# Autodesk Inventor assembly: Thrust_Duct
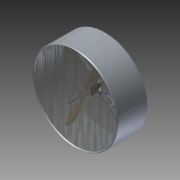
[picture p0: Inventor's stored thumbnail of the model, 180x180]
Saved by Autodesk Inventor 2011 SP1 (Build 150282100, 282)
## iProperties
Created: 2011-06-11
Part Number: Thrust_Duct
Document SubType Name: Assembly
Designer: Andrew G. Meyer
Mass: 210.395 g
Surface Area: 2926.53 cm^2
Volume: 210.395 cm^3
Density: 1 g/cm^3
Author: Andrew G. Meyer
## Documents named in this file (9)
- C:\Users\Andrew G. Meyer\Documents\Inventor\Hovercraft\Thrust_Duct.iam
- C:\Users\Andrew G. Meyer\Documents\Inventor\Hovercraft\Duct_Inner.ipt
- C:\Users\Andrew G. Meyer\Documents\Inventor\Hovercraft\Duct_Outer.ipt
- C:\Users\Andrew G. Meyer\Documents\Inventor\Hovercraft\Thrust_Support.ipt
- C:\Users\Andrew G. Meyer\Documents\Inventor\Hovercraft\Thrust_Motor.ipt
- C:\Users\Andrew G. Meyer\Documents\Inventor\Hovercraft\propellor.ipt
- C:\Users\Andrew G. Meyer\Documents\Inventor\Hovercraft\Duct_Guard.ipt
- C:\Users\Andrew G. Meyer\Documents\Inventor\Hovercraft\Thrust_Duct\AIP\Cable and Harness\Thrust_Duct_Harness.iam
- C:\Users\Andrew G. Meyer\Documents\Inventor\Hovercraft\ESC.ipt
## Components (11 placed, 8 different names)
1. Duct_Inner:1 — Mate:4, Insert:1, Insert:3
2. Duct_Outer:1 — Insert:3
3. Thrust_Support:1 — Mate:1, Flush:2, Mate:3, Flush:5, Flush:6
4. Thrust_Support:2 — Mate:1, Flush:2, Flush:4, Flush:6
5. Thrust_Support:3 — Mate:2, Flush:3, Mate:3, Flush:5, Mate:5, Mate:10
6. Thrust_Support:4 — Mate:2, Flush:3, Flush:4, Mate:4, Mate:8
7. Thrust_Motor:1 — Mate:5, Mate:6, Mate:7, Mate:8
8. propellor:1 — Mate:6, Mate:7
9. Duct_Guard:1 — Insert:1
10. Thrust_Duct_Harness [sub-assembly]
11. ESC:1 — Mate:10
## Relationships (16: Mate 9, Flush 5, Insert 2)
- Mate:1: Thrust_Support:1 ↔ Thrust_Support:2
- Flush:2: Thrust_Support:1 ↔ Thrust_Support:2
- Mate:2: Thrust_Support:3 ↔ Thrust_Support:4
- Flush:3: Thrust_Support:3 ↔ Thrust_Support:4
- Mate:3: Thrust_Support:1 ↔ Thrust_Support:3
- Flush:4: Thrust_Support:2 ↔ Thrust_Support:4
- Flush:5: Thrust_Support:1 ↔ Thrust_Support:3
- Flush:6: Thrust_Support:1 ↔ Thrust_Support:2
- Mate:4: Duct_Inner:1 ↔ Thrust_Support:4
- Mate:5: Thrust_Support:3 ↔ Thrust_Motor:1
- Mate:6: Thrust_Motor:1 ↔ propellor:1
- Mate:7: Thrust_Motor:1 ↔ propellor:1
- Mate:8: Thrust_Support:4 ↔ Thrust_Motor:1
- Insert:1: Duct_Inner:1 ↔ Duct_Guard:1
- Insert:3: Duct_Inner:1 ↔ Duct_Outer:1
- Mate:10: Thrust_Support:3 ↔ ESC:1
